# Autodesk Inventor assembly: Butterfly Drive Base
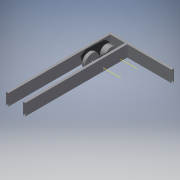
[picture p0: Inventor's stored thumbnail of the model, 180x180]
Saved by Autodesk Inventor 2019.4 (Build 234330000, 330)
## iProperties
Created: 2019-10-19
Part Number: Butterfly Drive Base
Document SubType Name: Assembly
Designer: Mark
Author: Mark
## Documents named in this file (6)
- C:\Users\admin\Desktop\FRC 2020 Engineering\GitHub\7738-CAD-prep\Butterfly drive\Butterfly Drive Base.iam
- C:\Users\admin\Desktop\FRC 2020 Engineering\GitHub\7738-CAD-prep\Butterfly drive\Butterfly Drive Module.iam
- C:\Users\admin\Desktop\FRC 2020 Engineering\GitHub\7738-CAD-prep\Butterfly drive\Side Extrusion.ipt
- C:\Users\admin\Desktop\FRC 2020 Engineering\GitHub\7738-CAD-prep\Butterfly drive\Module Plate 1.ipt
- C:\Users\admin\Desktop\FRC 2020 Engineering\GitHub\7738-CAD-prep\Butterfly drive\Side Extrusion 2.ipt
- C:\Users\admin\Desktop\FRC 2020 Engineering\GitHub\7738-CAD-prep\Butterfly drive\Back Extrusion 1.ipt
## Components (4 placed, 4 different names)
1. Butterfly Drive Module:1 [sub-assembly] — Mate:3, Mate:4, Mate:5, Angle:1
2. Side Extrusion:1 — Mate:1, Flush:1, Mate:5, Angle:1
3. Side Extrusion 2:1 — Flush:2, Mate:2, Flush:3, Mate:3, Mate:4, Mate:7
4. Back Extrusion 1:1 — Mate:1, Flush:1, Flush:2, Mate:2, Flush:3, Mate:6, Flush:4
## Relationships (12: Mate 7, Flush 4, Angle 1)
- Mate:1: Side Extrusion:1 ↔ Back Extrusion 1:1
- Flush:1: Side Extrusion:1 ↔ Back Extrusion 1:1
- Flush:2: Side Extrusion 2:1 ↔ Back Extrusion 1:1
- Mate:2: Side Extrusion 2:1 ↔ Back Extrusion 1:1
- Flush:3: Side Extrusion 2:1 ↔ Back Extrusion 1:1
- Mate:3: Butterfly Drive Module:1 ↔ Side Extrusion 2:1
- Mate:4 (0.3 mm): Butterfly Drive Module:1 ↔ Side Extrusion 2:1
- Mate:5 (5.3 mm): Butterfly Drive Module:1 ↔ Side Extrusion:1
- Mate:6: Back Extrusion 1:1
- Flush:4: Back Extrusion 1:1
- Mate:7: Side Extrusion 2:1
- Angle:1 (3 deg): Butterfly Drive Module:1 ↔ Side Extrusion:1
## Named parameters: Height = 80 mm, ExtSta = 0 deg, ModuleAngle = 3 deg
